# Autodesk Inventor assembly: подшипник внешнее кольцо с шариками
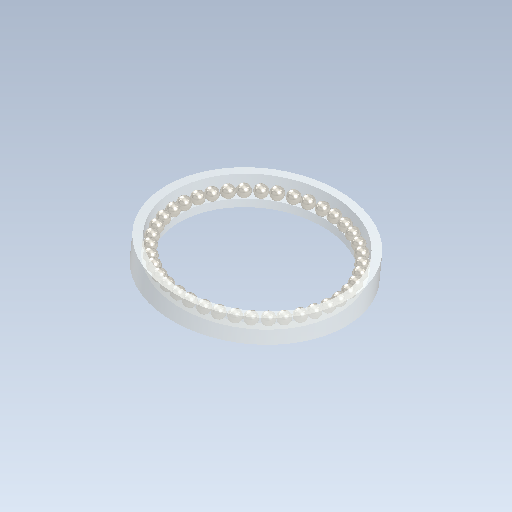
[picture p0: Inventor's stored thumbnail of the model, 512x512]
Saved by Autodesk Inventor 2020.1 (Build 241239000, 239)
## iProperties
Created: 2022-04-01
Part Number: подшипник внешнее кольцо с шариками
Document SubType Name: Assembly
Designer: User
Author: User
## Documents named in this file (3)
- D:\GitHub\TANK\3D-turret\подшипник внешнее кольцо с шариками.iam
- D:\GitHub\TANK\3D-turret\внешнее кольцо подшипника.ipt
- D:\GitHub\TANK\3D-turret\шарик подшипника.ipt
## Components (41 placed, 2 different names)
1. внешнее кольцо подшипника:1 — Касательность:1, Касательность:2, Касательность:3, Касательность:4
2. шарик подшипника:2 — Касательность:3, Касательность:4, Касательность:5
3. шарик подшипника:16 — Касательность:1, Касательность:2, Касательность:5
4. шарик подшипника:19
5. шарик подшипника:20
6. шарик подшипника:21
7. шарик подшипника:22
8. шарик подшипника:23
9. шарик подшипника:24
10. шарик подшипника:25
11. шарик подшипника:26
12. шарик подшипника:27
13. шарик подшипника:28
14. шарик подшипника:29
15. шарик подшипника:30
16. шарик подшипника:31
17. шарик подшипника:32
18. шарик подшипника:33
19. шарик подшипника:34
20. шарик подшипника:35
21. шарик подшипника:36
22. шарик подшипника:37
23. шарик подшипника:38
24. шарик подшипника:39
25. шарик подшипника:40
26. шарик подшипника:41
27. шарик подшипника:42
28. шарик подшипника:43
29. шарик подшипника:44
30. шарик подшипника:45
31. шарик подшипника:46
32. шарик подшипника:47
33. шарик подшипника:48
34. шарик подшипника:49
35. шарик подшипника:50
36. шарик подшипника:51
37. шарик подшипника:52
38. шарик подшипника:53
39. шарик подшипника:54
40. шарик подшипника:55
41. шарик подшипника:56
## Component patterns: (20 elements, first: шарик подшипника:2 + шарик подшипника:16)
## Relationships (5: Tangent 5)
- Касательность:1 [Tangent]: внешнее кольцо подшипника:1 ↔ шарик подшипника:16
- Касательность:2 [Tangent]: внешнее кольцо подшипника:1 ↔ шарик подшипника:16
- Касательность:3 [Tangent]: внешнее кольцо подшипника:1 ↔ шарик подшипника:2
- Касательность:4 [Tangent]: внешнее кольцо подшипника:1 ↔ шарик подшипника:2
- Касательность:5 [Tangent]: шарик подшипника:2 ↔ шарик подшипника:16
